# Autodesk Inventor assembly: Test tube rack
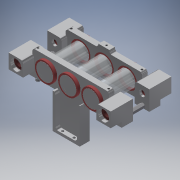
[picture p0: Inventor's stored thumbnail of the model, 180x180]
Saved by Autodesk Inventor 2017 (Build 210142000, 142)
## iProperties
Created: 2016-12-06
Part Number: Test tube rack
Document SubType Name: Assembly
Designer: qupec
Author: qupec
## Documents named in this file (12)
- C:\UMD\BPP\ROCKSAT X\STAR\CAD\Mechanical\Full payload assembly\Subsystems\Test Tube Rack\Test tube rack.iam
- C:\UMD\BPP\ROCKSAT X\STAR\CAD\Mechanical\Full payload assembly\Subsystems\Test Tube Rack\Test Tube Holder with Camera.ipt
- C:\UMD\BPP\ROCKSAT X\STAR\CAD\Mechanical\Full payload assembly\Subsystems\Test Tube Rack\Tube Rubber.ipt
- C:\UMD\BPP\ROCKSAT X\STAR\CAD\Mechanical\Full payload assembly\Subsystems\Test Tube Rack\Test Tube Holder.ipt
- C:\UMD\BPP\ROCKSAT X\STAR\CAD\Mechanical\Full payload assembly\Subsystems\Test Tube Rack\Bottom Test Tube Holder.ipt
- C:\UMD\BPP\ROCKSAT X\STAR\CAD\Mechanical\Full payload assembly\Subsystems\Test Tube Rack\Top Test Tube Holder.ipt
- C:\UMD\BPP\ROCKSAT X\STAR\CAD\Mechanical\Full payload assembly\Subsystems\Test Tube Rack\Self-Aligning PTFE Bearing.ipt
- C:\UMD\BPP\ROCKSAT X\STAR\CAD\Mechanical\Full payload assembly\Subsystems\Fasteners\Num4 Narrow Split Washer.ipt
- C:\UMD\BPP\ROCKSAT X\STAR\CAD\Mechanical\Full payload assembly\Subsystems\Fasteners\4-40 1in Socket Screw.ipt
- C:\UMD\BPP\ROCKSAT X\STAR\CAD\Mechanical\Full payload assembly\Subsystems\Fasteners\.75 in Standoff.ipt
- C:\UMD\BPP\ROCKSAT X\STAR\CAD\Mechanical\Full payload assembly\Subsystems\Fasteners\4-40 .625in Socket Screw.ipt
- C:\UMD\BPP\ROCKSAT X\STAR\CAD\Mechanical\Full payload assembly\Subsystems\Test Tube Rack\Test tube.iam
## Components (29 placed, 11 different names)
1. Test Tube Holder:1 — Mate:61, Mate:75, Mate:76, Mate:77, Mate:78, Mate:100, Mate:101, Mate:102, Mate:103, Flush:18, Mate:106, Mate:107, Mate:108, Mate:109, Mate:117
2. Bottom Test Tube Holder:1 — Mate:7, Mate:8, Mate:9, Mate:61, Mate:103, Mate:104, Mate:105
3. Tube Rubber:1 — Mate:104, Flush:19, Flush:20
4. Tube Rubber:2 — Mate:105, Flush:18, Flush:19
5. Tube Rubber:3 — Mate:8, Mate:82, Flush:16, Flush:17, Mate:119
6. Tube Rubber:4 — Mate:9, Flush:20
7. Tube Rubber:5 — Mate:7, Mate:83, Flush:15, Flush:16, Mate:120, Flush:21
8. Tube Rubber:6 — Mate:81, Flush:17, Mate:118
9. Test Tube Holder with Camera:1 — Mate:60, Mate:70, Flush:14, Mate:71, Mate:72, Mate:73, Mate:74, Mate:79, Mate:80, Mate:81, Flush:15, Mate:84, Mate:85, Mate:86, Mate:87, Mate:92, Mate:93, Mate:94, Mate:95, Mate:96, Mate:97, Mate:98, Mate:99, Mate:114
10. Top Test Tube Holder:1 — Mate:60, Mate:79, Mate:80, Mate:82, Mate:83
11. Self-Aligning PTFE Bearing:1 — Mate:71, Mate:74
12. Self-Aligning PTFE Bearing:2 — Mate:76, Mate:77
13. Self-Aligning PTFE Bearing:3 — Mate:75, Mate:78
14. Self-Aligning PTFE Bearing:4 — Mate:72, Mate:73
15. Num4 Narrow Split Washer:1 — Mate:84, Mate:85, Mate:115
16. Num4 Narrow Split Washer:2 — Mate:86, Mate:87, Mate:110, Mate:111
17. .75 in Standoff:1 — Mate:92, Mate:93, Mate:100
18. .75 in Standoff:2 — Mate:94, Mate:95, Mate:101, Mate:102
19. 4-40 .625in Socket Screw:1 — Mate:98, Mate:99
20. 4-40 .625in Socket Screw:2 — Mate:96, Mate:97
21. Num4 Narrow Split Washer:3 — Mate:106, Mate:107, Mate:116
22. Num4 Narrow Split Washer:4 — Mate:108, Mate:109, Mate:112, Mate:113
23. 4-40 1in Socket Screw:1 — Mate:110, Mate:111
24. 4-40 1in Socket Screw:2 — Mate:112, Mate:113
25. 4-40 1in Socket Screw:3 — Mate:116, Mate:117
26. 4-40 1in Socket Screw:4 — Mate:114, Mate:115
27. Test tube:1 [sub-assembly] — Mate:118, Flush:23
28. Test tube:2 [sub-assembly] — Mate:119, Flush:22, Flush:23
29. Test tube:3 [sub-assembly] — Mate:120, Flush:21, Flush:22
## Relationships (62: Mate 52, Flush 10)
- Mate:7: Bottom Test Tube Holder:1 ↔ Tube Rubber:5
- Mate:8: Bottom Test Tube Holder:1 ↔ Tube Rubber:3
- Mate:9: Bottom Test Tube Holder:1 ↔ Tube Rubber:4
- Mate:60: Test Tube Holder with Camera:1 ↔ Top Test Tube Holder:1
- Mate:61: Test Tube Holder:1 ↔ Bottom Test Tube Holder:1
- Mate:70: Test Tube Holder with Camera:1
- Flush:14: Test Tube Holder with Camera:1
- Mate:71: Test Tube Holder with Camera:1 ↔ Self-Aligning PTFE Bearing:1
- Mate:72: Test Tube Holder with Camera:1 ↔ Self-Aligning PTFE Bearing:4
- Mate:73: Test Tube Holder with Camera:1 ↔ Self-Aligning PTFE Bearing:4
- Mate:74: Test Tube Holder with Camera:1 ↔ Self-Aligning PTFE Bearing:1
- Mate:75: Test Tube Holder:1 ↔ Self-Aligning PTFE Bearing:3
- Mate:76: Test Tube Holder:1 ↔ Self-Aligning PTFE Bearing:2
- Mate:77: Test Tube Holder:1 ↔ Self-Aligning PTFE Bearing:2
- Mate:78: Test Tube Holder:1 ↔ Self-Aligning PTFE Bearing:3
- Mate:79: Test Tube Holder with Camera:1 ↔ Top Test Tube Holder:1
- Mate:80: Test Tube Holder with Camera:1 ↔ Top Test Tube Holder:1
- Mate:81: Tube Rubber:6 ↔ Test Tube Holder with Camera:1
- Mate:82: Tube Rubber:3 ↔ Top Test Tube Holder:1
- Mate:83: Tube Rubber:5 ↔ Top Test Tube Holder:1
- Flush:15: Tube Rubber:5 ↔ Test Tube Holder with Camera:1
- Flush:16: Tube Rubber:3 ↔ Tube Rubber:5
- Flush:17: Tube Rubber:3 ↔ Tube Rubber:6
- Mate:84: Test Tube Holder with Camera:1 ↔ Num4 Narrow Split Washer:1
- Mate:85: Test Tube Holder with Camera:1 ↔ Num4 Narrow Split Washer:1
- Mate:86: Test Tube Holder with Camera:1 ↔ Num4 Narrow Split Washer:2
- Mate:87: Test Tube Holder with Camera:1 ↔ Num4 Narrow Split Washer:2
- Mate:92: Test Tube Holder with Camera:1 ↔ .75 in Standoff:1
- Mate:93: Test Tube Holder with Camera:1 ↔ .75 in Standoff:1
- Mate:94: Test Tube Holder with Camera:1 ↔ .75 in Standoff:2
- Mate:95: Test Tube Holder with Camera:1 ↔ .75 in Standoff:2
- Mate:96: Test Tube Holder with Camera:1 ↔ 4-40 .625in Socket Screw:2
- Mate:97: Test Tube Holder with Camera:1 ↔ 4-40 .625in Socket Screw:2
- Mate:98: Test Tube Holder with Camera:1 ↔ 4-40 .625in Socket Screw:1
- Mate:99: Test Tube Holder with Camera:1 ↔ 4-40 .625in Socket Screw:1
- Mate:100: Test Tube Holder:1 ↔ .75 in Standoff:1
- Mate:101: Test Tube Holder:1 ↔ .75 in Standoff:2
- Mate:102: Test Tube Holder:1 ↔ .75 in Standoff:2
- Mate:103: Test Tube Holder:1 ↔ Bottom Test Tube Holder:1
- Mate:104: Bottom Test Tube Holder:1 ↔ Tube Rubber:1
- Mate:105: Bottom Test Tube Holder:1 ↔ Tube Rubber:2
- Flush:18: Test Tube Holder:1 ↔ Tube Rubber:2
- Flush:19: Tube Rubber:1 ↔ Tube Rubber:2
- Flush:20: Tube Rubber:1 ↔ Tube Rubber:4
- Mate:106: Test Tube Holder:1 ↔ Num4 Narrow Split Washer:3
- Mate:107: Test Tube Holder:1 ↔ Num4 Narrow Split Washer:3
- Mate:108: Test Tube Holder:1 ↔ Num4 Narrow Split Washer:4
- Mate:109: Test Tube Holder:1 ↔ Num4 Narrow Split Washer:4
- Mate:110: Num4 Narrow Split Washer:2 ↔ 4-40 1in Socket Screw:1
- Mate:111: Num4 Narrow Split Washer:2 ↔ 4-40 1in Socket Screw:1
- Mate:112: Num4 Narrow Split Washer:4 ↔ 4-40 1in Socket Screw:2
- Mate:113: Num4 Narrow Split Washer:4 ↔ 4-40 1in Socket Screw:2
- Mate:114: Test Tube Holder with Camera:1 ↔ 4-40 1in Socket Screw:4
- Mate:115: Num4 Narrow Split Washer:1 ↔ 4-40 1in Socket Screw:4
- Mate:116: Num4 Narrow Split Washer:3 ↔ 4-40 1in Socket Screw:3
- Mate:117: Test Tube Holder:1 ↔ 4-40 1in Socket Screw:3
- Mate:118: Tube Rubber:6 ↔ Test tube:1
- Mate:119: Tube Rubber:3 ↔ Test tube:2
- Mate:120: Tube Rubber:5 ↔ Test tube:3
- Flush:21: Tube Rubber:5 ↔ Test tube:3
- Flush:22: Test tube:2 ↔ Test tube:3
- Flush:23: Test tube:1 ↔ Test tube:2
